# Autodesk Inventor assembly: Front Z Axis
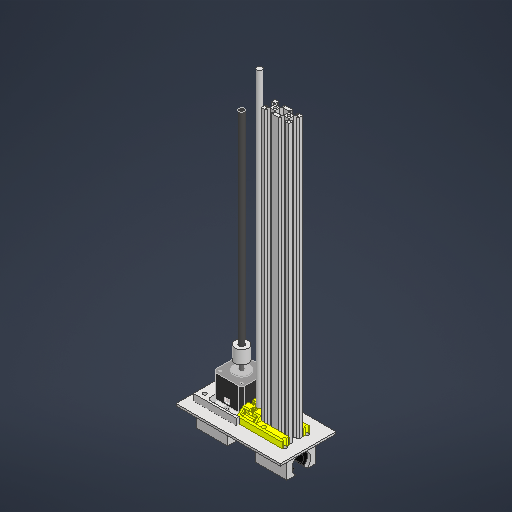
[picture p0: Inventor's stored thumbnail of the model, 512x512]
Saved by Autodesk Inventor 2025.1 (Build 291241000, 241)
## iProperties
Created: 2024-11-25
Part Number: Front Z Axis
Document SubType Name: Assembly
Designer: jerem
Author: jerem
## Documents named in this file (11)
- C:\Users\jerem\Documents\GitHub\Perovskite-Automated-Synthesis-System\CAD\Gantry\Front Z Axis\Front Z Axis.iam
- C:\Users\jerem\Documents\GitHub\Perovskite-Automated-Synthesis-System\CAD\Non 3D Printed Parts\X Axis Base Plate.ipt
- C:\Users\jerem\Documents\GitHub\Perovskite-Automated-Synthesis-System\CAD\Gantry\Rot Bottom Mount.ipt
- C:\Users\jerem\Documents\GitHub\Perovskite-Automated-Synthesis-System\CAD\Non 3D Printed Parts\Linear Rails\8mm Linear Rod.ipt
- C:\Users\jerem\Documents\GitHub\Perovskite-Automated-Synthesis-System\CAD\Non 3D Printed Parts\Motors and Servos\NEMA17 Stepper Motor.ipt
- C:\Users\jerem\Documents\GitHub\Perovskite-Automated-Synthesis-System\CAD\Non 3D Printed Parts\Threaded Rod 300mm.ipt
- C:\Users\jerem\Documents\GitHub\Perovskite-Automated-Synthesis-System\CAD\Non 3D Printed Parts\Rod Coupler.ipt
- C:\Users\jerem\Documents\GitHub\Perovskite-Automated-Synthesis-System\CAD\Non 3D Printed Parts\Extrusion\V Extrustion 40x400mm.ipt
- C:\Users\jerem\Documents\GitHub\Perovskite-Automated-Synthesis-System\CAD\Non 3D Printed Parts\Linear Rails\Linear Rail Slider Block.ipt
- C:\Users\jerem\Documents\GitHub\Perovskite-Automated-Synthesis-System\CAD\Non 3D Printed Parts\Screws\M5x12.ipt
- C:\Users\jerem\Documents\GitHub\Perovskite-Automated-Synthesis-System\CAD\Gantry\Stepper Z Mount.ipt
## Components (12 placed, 10 different names)
1. X Axis Base Plate:1 — Mate:13, Mate:14, Mate:15, Mate:16, Mate:17, Mate:18, Mate:19, Mate:23, Mate:24, Mate:26, Mate:27, Mate:29, Mate:30
2. V Extrustion 40x400mm:1
3. NEMA17 Stepper Motor:1 — Mate:28
4. Threaded Rod 300mm:1
5. Rod Coupler:1
6. Rot Bottom Mount:1 — Mate:19, Mate:28
7. 8mm Linear Rod:1
8. Linear Rail Slider Block:1 — Mate:13, Mate:16, Mate:17
9. Linear Rail Slider Block:2 — Mate:14, Mate:15, Mate:18
10. M5x12:2 — Mate:23, Mate:27
11. M5x12:3 — Mate:24, Mate:26
12. Stepper Z Mount:1 — Mate:29, Mate:30
## Relationships (26: Mate 25, Angle 1)
- [Mate]: X Axis Base Plate:1 ↔ V Extrustion 40x400mm:1
- [Angle] (0 deg): X Axis Base Plate:1 ↔ V Extrustion 40x400mm:1
- [Mate]: NEMA17 Stepper Motor:1 ↔ Rod Coupler:1
- [Mate]: Threaded Rod 300mm:1 ↔ Rod Coupler:1
- [Mate] (-8 mm): NEMA17 Stepper Motor:1 ↔ Rod Coupler:1
- [Mate] (-8 mm): Threaded Rod 300mm:1 ↔ Rod Coupler:1
- [Mate]: X Axis Base Plate:1 ↔ Rot Bottom Mount:1
- [Mate]: Rot Bottom Mount:1 ↔ 8mm Linear Rod:1
- [Mate]: X Axis Base Plate:1 ↔ 8mm Linear Rod:1
- [Mate]: NEMA17 Stepper Motor:1 ↔ Rot Bottom Mount:1
- [Mate]: V Extrustion 40x400mm:1 ↔ Rot Bottom Mount:1
- [Mate]: V Extrustion 40x400mm:1 ↔ Rot Bottom Mount:1
- Mate:13: X Axis Base Plate:1 ↔ Linear Rail Slider Block:1
- Mate:14: X Axis Base Plate:1 ↔ Linear Rail Slider Block:2
- Mate:15: X Axis Base Plate:1 ↔ Linear Rail Slider Block:2
- Mate:16: X Axis Base Plate:1 ↔ Linear Rail Slider Block:1
- Mate:17: X Axis Base Plate:1 ↔ Linear Rail Slider Block:1
- Mate:18: X Axis Base Plate:1 ↔ Linear Rail Slider Block:2
- Mate:19: X Axis Base Plate:1 ↔ Rot Bottom Mount:1
- Mate:23: X Axis Base Plate:1 ↔ M5x12:2
- Mate:24: X Axis Base Plate:1 ↔ M5x12:3
- Mate:26: X Axis Base Plate:1 ↔ M5x12:3
- Mate:27: X Axis Base Plate:1 ↔ M5x12:2
- Mate:28: NEMA17 Stepper Motor:1 ↔ Rot Bottom Mount:1
- Mate:29: X Axis Base Plate:1 ↔ Stepper Z Mount:1
- Mate:30: X Axis Base Plate:1 ↔ Stepper Z Mount:1
